# Autodesk Inventor assembly: ASSEMBLY_Main
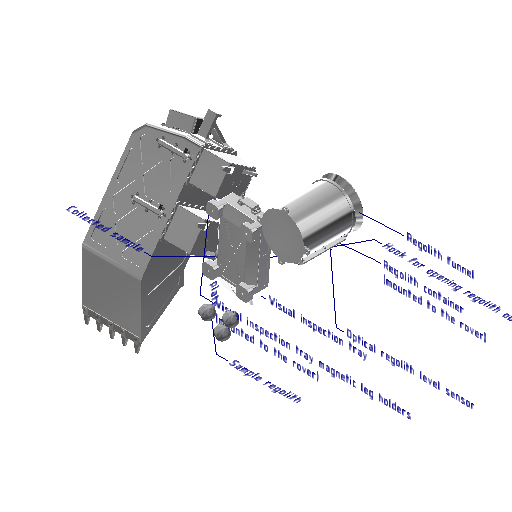
[picture p0: Inventor's stored thumbnail of the model, 512x512]
Saved by Autodesk Inventor 2025 (Build 290162010, 162A)
## iProperties
Created: 2018-09-12
Part Number: ASSEMBLY_Main
Document SubType Name: Assembly
Designer: Andrzej
Mass: 460.401 g
Surface Area: 1990.25 cm^2
Volume: 164.779 cm^3
Density: 2.79405 g/cm^3
Author: Andrzej
## Documents named in this file (15)
- D:\_ANDRZEJ_LACZEWSKI\_OTHER\MECH - My entry for the NASA Lunar Sampling System Design Challenge\MCAD\1_REV1\ASSEMBLY_MAIN_REVA\ASSEMBLY_Main.iam
- D:\_ANDRZEJ_LACZEWSKI\_OTHER\MECH - My entry for the NASA Lunar Sampling System Design Challenge\MCAD\1_REV1\ASSEMBLY_MAIN_REVA\CNCM_ALU_Sorting_shovel_base_plate.ipt
- D:\_ANDRZEJ_LACZEWSKI\_OTHER\MECH - My entry for the NASA Lunar Sampling System Design Challenge\MCAD\1_REV1\ASSEMBLY_MAIN_REVA\CNCM_ALU_Second_sieve.ipt
- D:\_ANDRZEJ_LACZEWSKI\_OTHER\MECH - My entry for the NASA Lunar Sampling System Design Challenge\MCAD\1_REV1\ASSEMBLY_MAIN_REVA\CNCM_ALU_Sorting_shovel_top_plate.ipt
- D:\_ANDRZEJ_LACZEWSKI\_OTHER\MECH - My entry for the NASA Lunar Sampling System Design Challenge\MCAD\1_REV1\ASSEMBLY_MAIN_REVA\CNCM_ALU_First_barrier.ipt
- D:\_ANDRZEJ_LACZEWSKI\_OTHER\MECH - My entry for the NASA Lunar Sampling System Design Challenge\MCAD\1_REV1\ASSEMBLY_MAIN_REVA\CNCM_ALU_First_sieve.ipt
- D:\_ANDRZEJ_LACZEWSKI\_OTHER\MECH - My entry for the NASA Lunar Sampling System Design Challenge\MCAD\1_REV1\ASSEMBLY_MAIN_REVA\ASSEMBLY_Vibration_module.iam
- D:\_ANDRZEJ_LACZEWSKI\_OTHER\MECH - My entry for the NASA Lunar Sampling System Design Challenge\MCAD\1_REV1\ASSEMBLY_MAIN_REVA\ASSEMBLY_Regolith_level_sensor_with_screws.iam
- D:\_ANDRZEJ_LACZEWSKI\_OTHER\MECH - My entry for the NASA Lunar Sampling System Design Challenge\MCAD\1_REV1\ASSEMBLY_MAIN_REVA\ASSEMBLY_Bucket_tooth.iam
- D:\_ANDRZEJ_LACZEWSKI\_OTHER\MECH - My entry for the NASA Lunar Sampling System Design Challenge\MCAD\1_REV1\ASSEMBLY_MAIN_REVA\ASSEMBLY_Regolith_Container.iam
- D:\_ANDRZEJ_LACZEWSKI\_OTHER\MECH - My entry for the NASA Lunar Sampling System Design Challenge\MCAD\1_REV1\ASSEMBLY_MAIN_REVA\ASSEMBLY_Visual_inspection_tray.iam
- D:\_ANDRZEJ_LACZEWSKI\_OTHER\MECH - My entry for the NASA Lunar Sampling System Design Challenge\MCAD\1_REV1\ASSEMBLY_MAIN_REVA\CNCM_ALU_Visual_inspection_tray_hook.ipt
- D:\_ANDRZEJ_LACZEWSKI\_OTHER\MECH - My entry for the NASA Lunar Sampling System Design Challenge\MCAD\1_REV1\ASSEMBLY_MAIN_REVA\ASSEMBLY_Outlet_channel_1.iam
- D:\_ANDRZEJ_LACZEWSKI\_OTHER\MECH - My entry for the NASA Lunar Sampling System Design Challenge\MCAD\1_REV1\ASSEMBLY_MAIN_REVA\ASSEMBLY_Outlet_channel_2.iam
- D:\_ANDRZEJ_LACZEWSKI\_OTHER\MECH - My entry for the NASA Lunar Sampling System Design Challenge\MCAD\1_REV1\ASSEMBLY_MAIN_REVA\OTH_15mm_rock.ipt
## Components (19 placed, 14 different names)
1. CNCM_ALU_Sorting_shovel_base_plate:1 — Mate:3, Mate:4, Mate:5, Mate:17, Mate:23, Mate:24, Mate:26, Mate:27, Mate:28, Flush:8, Flush:9, Flush:10, Mate:35, Mate:36, Mate:43, Mate:45, Mate:46, Mate:47, Mate:48, Mate:49, Mate:50, Mate:51, Mate:52, Mate:53, Mate:59, Mate:60, Flush:16, Mate:63, Mate:64, Flush:19, Flush:20, Flush:21, Flush:22, Mate:65, Mate:66, Mate:67, Mate:68
2. CNCM_ALU_Second_sieve:1 — Mate:3, Mate:4, Mate:5, Mate:25
3. CNCM_ALU_First_barrier:1 — Mate:17, Mate:28, Flush:9
4. CNCM_ALU_First_sieve:1 — Mate:23, Mate:24, Mate:25
5. CNCM_ALU_First_barrier:2 — Mate:26, Mate:27, Flush:8
6. CNCM_ALU_Sorting_shovel_top_plate:1 — Flush:10, Mate:35, Mate:36
7. ASSEMBLY_Vibration_module:1 [sub-assembly] — Mate:43, Mate:65, Mate:66
8. ASSEMBLY_Regolith_level_sensor_with_screws:1 [sub-assembly] — Mate:46, Mate:47, Mate:50
9. ASSEMBLY_Regolith_level_sensor_with_screws:2 [sub-assembly] — Mate:45, Mate:48, Mate:49
10. ASSEMBLY_Bucket_tooth:1 [sub-assembly] — Mate:51, Mate:52, Mate:53
11. CNCM_ALU_Visual_inspection_tray_hook:1 — Mate:59, Mate:60, Flush:16
12. ASSEMBLY_Outlet_channel_2:1 [sub-assembly] — Mate:64, Flush:19, Flush:20
13. ASSEMBLY_Outlet_channel_1:1 [sub-assembly] — Mate:63, Flush:21, Flush:22
14. ASSEMBLY_Regolith_Container:1 [sub-assembly] — Flush:24, Mate:69
15. ASSEMBLY_Visual_inspection_tray:1 [sub-assembly] — Flush:24
16. OTH_15mm_rock:2
17. OTH_15mm_rock:3
18. OTH_15mm_rock:4
19. OTH_15mm_rock:5
## Relationships (40: Mate 31, Flush 9)
- Mate:3: CNCM_ALU_Sorting_shovel_base_plate:1 ↔ CNCM_ALU_Second_sieve:1
- Mate:4: CNCM_ALU_Sorting_shovel_base_plate:1 ↔ CNCM_ALU_Second_sieve:1
- Mate:5 (50 mm): CNCM_ALU_Sorting_shovel_base_plate:1 ↔ CNCM_ALU_Second_sieve:1
- Mate:17: CNCM_ALU_Sorting_shovel_base_plate:1 ↔ CNCM_ALU_First_barrier:1
- Mate:23: CNCM_ALU_Sorting_shovel_base_plate:1 ↔ CNCM_ALU_First_sieve:1
- Mate:24: CNCM_ALU_Sorting_shovel_base_plate:1 ↔ CNCM_ALU_First_sieve:1
- Mate:25 (50 mm): CNCM_ALU_Second_sieve:1 ↔ CNCM_ALU_First_sieve:1
- Mate:26: CNCM_ALU_Sorting_shovel_base_plate:1 ↔ CNCM_ALU_First_barrier:2
- Mate:27: CNCM_ALU_Sorting_shovel_base_plate:1 ↔ CNCM_ALU_First_barrier:2
- Mate:28: CNCM_ALU_Sorting_shovel_base_plate:1 ↔ CNCM_ALU_First_barrier:1
- Flush:8: CNCM_ALU_Sorting_shovel_base_plate:1 ↔ CNCM_ALU_First_barrier:2
- Flush:9: CNCM_ALU_Sorting_shovel_base_plate:1 ↔ CNCM_ALU_First_barrier:1
- Flush:10: CNCM_ALU_Sorting_shovel_base_plate:1 ↔ CNCM_ALU_Sorting_shovel_top_plate:1
- Mate:35: CNCM_ALU_Sorting_shovel_base_plate:1 ↔ CNCM_ALU_Sorting_shovel_top_plate:1
- Mate:36: CNCM_ALU_Sorting_shovel_base_plate:1 ↔ CNCM_ALU_Sorting_shovel_top_plate:1
- Mate:43: CNCM_ALU_Sorting_shovel_base_plate:1 ↔ ASSEMBLY_Vibration_module:1
- Mate:45: CNCM_ALU_Sorting_shovel_base_plate:1 ↔ ASSEMBLY_Regolith_level_sensor_with_screws:2
- Mate:46: CNCM_ALU_Sorting_shovel_base_plate:1 ↔ ASSEMBLY_Regolith_level_sensor_with_screws:1
- Mate:47: CNCM_ALU_Sorting_shovel_base_plate:1 ↔ ASSEMBLY_Regolith_level_sensor_with_screws:1
- Mate:48: CNCM_ALU_Sorting_shovel_base_plate:1 ↔ ASSEMBLY_Regolith_level_sensor_with_screws:2
- Mate:49: CNCM_ALU_Sorting_shovel_base_plate:1 ↔ ASSEMBLY_Regolith_level_sensor_with_screws:2
- Mate:50: CNCM_ALU_Sorting_shovel_base_plate:1 ↔ ASSEMBLY_Regolith_level_sensor_with_screws:1
- Mate:51: CNCM_ALU_Sorting_shovel_base_plate:1 ↔ ASSEMBLY_Bucket_tooth:1
- Mate:52: CNCM_ALU_Sorting_shovel_base_plate:1 ↔ ASSEMBLY_Bucket_tooth:1
- Mate:53: CNCM_ALU_Sorting_shovel_base_plate:1 ↔ ASSEMBLY_Bucket_tooth:1
- Mate:59: CNCM_ALU_Sorting_shovel_base_plate:1 ↔ CNCM_ALU_Visual_inspection_tray_hook:1
- Mate:60: CNCM_ALU_Sorting_shovel_base_plate:1 ↔ CNCM_ALU_Visual_inspection_tray_hook:1
- Flush:16: CNCM_ALU_Sorting_shovel_base_plate:1 ↔ CNCM_ALU_Visual_inspection_tray_hook:1
- Mate:63: CNCM_ALU_Sorting_shovel_base_plate:1 ↔ ASSEMBLY_Outlet_channel_1:1
- Mate:64: CNCM_ALU_Sorting_shovel_base_plate:1 ↔ ASSEMBLY_Outlet_channel_2:1
- Flush:19: CNCM_ALU_Sorting_shovel_base_plate:1 ↔ ASSEMBLY_Outlet_channel_2:1
- Flush:20: CNCM_ALU_Sorting_shovel_base_plate:1 ↔ ASSEMBLY_Outlet_channel_2:1
- Flush:21: CNCM_ALU_Sorting_shovel_base_plate:1 ↔ ASSEMBLY_Outlet_channel_1:1
- Flush:22: CNCM_ALU_Sorting_shovel_base_plate:1 ↔ ASSEMBLY_Outlet_channel_1:1
- Mate:65: CNCM_ALU_Sorting_shovel_base_plate:1 ↔ ASSEMBLY_Vibration_module:1
- Mate:66: CNCM_ALU_Sorting_shovel_base_plate:1 ↔ ASSEMBLY_Vibration_module:1
- Flush:24: ASSEMBLY_Regolith_Container:1 ↔ ASSEMBLY_Visual_inspection_tray:1
- Mate:67: CNCM_ALU_Sorting_shovel_base_plate:1
- Mate:68: CNCM_ALU_Sorting_shovel_base_plate:1
- Mate:69: ASSEMBLY_Regolith_Container:1
